# Autodesk Inventor assembly: Assembly2
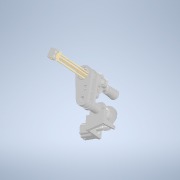
[picture p0: Inventor's stored thumbnail of the model, 180x180]
Saved by Autodesk Inventor 2020 (Build 240168000, 168)
## iProperties
Created: 2019-05-26
Part Number: Assembly2
Document SubType Name: Assembly
Designer: isadmin
Author: isadmin
## Documents named in this file (14)
- C:\Users\isadmin\Documents\Inventor\IS_2019June01\Assembly2.iam
- Assembly_ISv01.iam
- C:\Users\isadmin\Documents\Inventor\IS_2019June01\Shield_1.ipt
- C:\Users\isadmin\Documents\Inventor\IS_2019June01\block.ipt
- C:\Users\isadmin\Documents\Inventor\IS_2019June01\Shutter.ipt
- C:\Users\isadmin\Documents\Inventor\IS_2019June01\ceramic washer.ipt
- C:\Users\isadmin\Documents\Inventor\IS_2019June01\Shielding.ipt
- C:\Users\isadmin\Documents\Inventor\IS_2019June01\Bullet_v5_SiliconeSample.ipt
- C:\Users\isadmin\Documents\Inventor\IS_2019June01\Bullet_v5_SiliconeSample_TopPart.ipt
- C:\Users\isadmin\Documents\Inventor\IS_2019June01\670000.ipt
- C:\Users\isadmin\Documents\Inventor\IS_2019June01\MCF275-FlgMplxr-Cr1A5_(53-321020-A).ipt
- C:\Users\isadmin\Documents\Inventor\IS_2019June01\665501.ipt
- C:\Users\isadmin\Documents\Inventor\IS_2019June01\Shield_1 - Copy.ipt
- C:\Users\isadmin\Documents\Inventor\IS_2019June01\FlangeCF275 Bored_1112112 REV 1 .ipt
## Components (19 placed, 12 different names)
1. rotatable rod table:1 — Insert:6, Mate:23, Insert:8
2. block for bullet:1
3. Shutter:1
4. ceramic washer:1
5. ceramic washer:2
6. ceramic washer:3
7. ceramic washer:4
8. Shielding:1
9. ceramic washer:5
10. ceramic washer:6
11. ceramic washer:7
12. ceramic washer:8
13. Bullet_v5_SiliconeSample:1
14. Bullet_v5_SiliconeSample_TopPart:1
15. rotation_670000:1 — Insert:6
16. MCF275-FlgMplxr-Cr1A5_(53-321020-A):1 — Insert:5
17. zstage_665501:1 — Insert:7
18. moving tabe 4 rod:1 — Mate:23, Insert:8
19. FlangeCF275 Bored_1112112 REV 1 :1 — Insert:7, Insert:5
## Relationships (33: Mate 23, Insert 8, Flush 2)
- [Mate]: block for bullet:1 ↔ Shutter:1
- [Mate]: block for bullet:1 ↔ Shutter:1
- [Mate]: block for bullet:1 ↔ Shutter:1
- [Mate]: block for bullet:1 ↔ ceramic washer:2
- [Mate]: block for bullet:1 ↔ ceramic washer:2
- [Mate]: block for bullet:1 ↔ ceramic washer:1
- [Mate]: block for bullet:1 ↔ ceramic washer:1
- [Mate]: block for bullet:1 ↔ ceramic washer:4
- [Mate]: block for bullet:1 ↔ ceramic washer:4
- [Mate]: block for bullet:1 ↔ ceramic washer:3
- [Mate]: block for bullet:1 ↔ ceramic washer:3
- [Mate]: ceramic washer:1 ↔ Shielding:1
- [Flush]: block for bullet:1 ↔ Shielding:1
- [Flush]: block for bullet:1 ↔ Shielding:1
- [Mate]: block for bullet:1 ↔ ceramic washer:5
- [Mate]: block for bullet:1 ↔ ceramic washer:5
- [Mate]: block for bullet:1 ↔ ceramic washer:6
- [Mate]: block for bullet:1 ↔ ceramic washer:6
- [Mate]: block for bullet:1 ↔ ceramic washer:7
- [Mate]: block for bullet:1 ↔ ceramic washer:7
- [Mate]: block for bullet:1 ↔ ceramic washer:8
- [Mate]: block for bullet:1 ↔ ceramic washer:8
- [Mate] (0.0254 mm): Bullet_v5_SiliconeSample:1 ↔ Bullet_v5_SiliconeSample_TopPart:1
- [Mate]: Bullet_v5_SiliconeSample:1 ↔ Bullet_v5_SiliconeSample_TopPart:1
- [Insert]: block for bullet:1 ↔ Bullet_v5_SiliconeSample:1
- [Insert]: rotatable rod table:1 ↔ block for bullet:1
- [Insert]: rotatable rod table:1 ↔ block for bullet:1
- [Insert] (-0.254 mm): rotation_670000:1 ↔ MCF275-FlgMplxr-Cr1A5_(53-321020-A):1
- Insert:5 (-0.381 mm): MCF275-FlgMplxr-Cr1A5_(53-321020-A):1 ↔ FlangeCF275 Bored_1112112 REV 1 :1
- Insert:6: rotatable rod table:1 ↔ rotation_670000:1
- Insert:7 (0.381 mm): zstage_665501:1 ↔ FlangeCF275 Bored_1112112 REV 1 :1
- Mate:23: rotatable rod table:1 ↔ moving tabe 4 rod:1
- Insert:8: rotatable rod table:1 ↔ moving tabe 4 rod:1
## Named parameters: d75_d58 = 0 mm, d76_d19 = 0 mm, d77_d22_d25 = 0 mm, d78_d23_d26 = 0 mm, d79_d24_d35 = 0 mm, d80_d25_d36 = 0 mm, d81_d26_d37 = 0 mm, d82_d27_d38 = 0 mm, d83_d28_d39 = 0 mm, d84_d29_d40 = 0 mm, d85_d30_d41 = 0 mm, d86_d31_d42 = 0 mm, d87_d43 = 0 mm, d88_d44 = 0 mm, d89_d45 = 0 mm, d90_d46 = 0 mm, d91_d47 = 0 mm, d92_d48 = 0 mm, d93_d49 = 0 mm, d94_d50 = 0 mm, d95_d51 = 0 mm, d96_d52 = 0 mm, d97_d53 = 0 mm, d98_d56_d0 = 0.0254 mm, d99_d57_d1 = 0 mm
